# Autodesk Inventor assembly: SAR330  x 5 front + limit switches
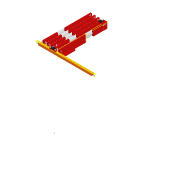
[picture p0: Inventor's stored thumbnail of the model, 180x180]
Saved by Autodesk Inventor 2020 (Build 240168000, 168)
## iProperties
Created: 2019-11-17
Part Number: SAR330  x 5 front + limit switches
Document SubType Name: Assembly
Designer: ball
Author: ball
## Documents named in this file (14)
- C:\FTC\FTC8863CAD\2019 Robot\Delivery\SAR330  x 5 front + limit switches.iam
- C:\FTC\FTC8863CAD\2019 Robot\Delivery\SAR330  x 5 + front couplers.iam
- C:\FTC\FTC8863CAD\Actobotics\605 parts\605630.ipt
- C:\FTC\FTC8863CAD\2019 Robot\Delivery\Coupler receiver.ipt
- C:\FTC\FTC8863CAD\RevRobotics\REV-41-1017_15mm_extrusion_17.875in.ipt
- C:\FTC\FTC8863CAD\StepLibraries\Screws\M3x6 SOCKET HEAD CAP SCREW.ipt
- C:\FTC\FTC8863CAD\2019 Robot\Delivery\Limit switch mount top.ipt
- C:\FTC\FTC8863CAD\2019 Robot\Delivery\Limit swtich mount bottom.ipt
- C:\FTC\FTC8863CAD\StepLibraries\Nuts\2-56 NYLON-INSERT LOCKNUT.ipt
- C:\FTC\FTC8863CAD\StepLibraries\Screws\2-56 x 0_5 SOCKET HEAD CAP SCREW.ipt
- C:\FTC\FTC8863CAD\StepLibraries\Nuts\m3 18-8 STAINLESS STL NYLON-INSERT LOCKNUT.ipt
- C:\FTC\FTC8863CAD\StepLibraries\Screws\M3 x 12 HEX HEAD CAP SCREW.ipt
- C:\FTC\FTC8863CAD\StepLibraries\Screws\M3 x 25 HEX HEAD CAP SCREW.ipt
- C:\FTC\FTC8863CAD\2019 Robot\Delivery\Limit switch mount top front.ipt
## Components (19 placed, 13 different names)
1. SAR330  x 5 + front couplers:1 [sub-assembly] — Flush:1, Flush:2, Mate:1, Mate:2, Flush:3, Flush:4, Mate:3, Flush:5, Flush:6, Mate:5, Flush:7, Mate:6, Flush:8, Flush:9, Mate:18, Mate:19, Flush:13, Mate:20, Flush:14, Flush:15
2. 605630:1 — Flush:1, Flush:2, Mate:1
3. Coupler receiver:1 — Mate:2, Flush:3, Flush:4
4. REV-41-1017_15mm_extrusion_17.875in:1 — Mate:3, Flush:5, Flush:6, Mate:4, Flush:10, Flush:11, Flush:12, Mate:16
5. 605630:2 — Mate:4, Mate:5, Flush:7, Mate:9, Mate:10, Mate:11
6. M3x6 SOCKET HEAD CAP SCREW:3 — Mate:6
7. Limit switch mount top:1 — Flush:8, Flush:9
8. Limit swtich mount bottom:1 — Flush:10, Flush:11, Flush:12, Mate:8, Mate:12, Mate:13, Mate:14, Mate:15
9. 2-56 NYLON-INSERT LOCKNUT:1
10. 2-56 NYLON-INSERT LOCKNUT:2 — Mate:8, Mate:9
11. 2-56 x 0_5 SOCKET HEAD CAP SCREW:1 — Mate:10, Mate:11
12. m3 18-8 STAINLESS STL NYLON-INSERT LOCKNUT:1 — Mate:12, Mate:13, Mate:17
13. m3 18-8 STAINLESS STL NYLON-INSERT LOCKNUT:2 — Mate:14, Mate:15
14. M3 x 12 HEX HEAD CAP SCREW:1 — Mate:16, Mate:17
15. 605630:3 — Flush:13, Mate:20, Flush:14, Mate:21, Mate:24
16. M3 x 25 HEX HEAD CAP SCREW:1 — Mate:18, Mate:19
17. Limit switch mount top front:1 — Flush:15, Mate:22
18. 2-56 x 0_5 SOCKET HEAD CAP SCREW:2 — Mate:21, Mate:22, Mate:23
19. 2-56 NYLON-INSERT LOCKNUT:3 — Mate:23, Mate:24
## Relationships (39: Mate 24, Flush 15)
- Flush:1 (14.605 mm): SAR330  x 5 + front couplers:1 ↔ 605630:1
- Flush:2 (10.16 mm): SAR330  x 5 + front couplers:1 ↔ 605630:1
- Mate:1 (2.8702 mm): SAR330  x 5 + front couplers:1 ↔ 605630:1
- Mate:2: SAR330  x 5 + front couplers:1 ↔ Coupler receiver:1
- Flush:3: SAR330  x 5 + front couplers:1 ↔ Coupler receiver:1
- Flush:4: SAR330  x 5 + front couplers:1 ↔ Coupler receiver:1
- Mate:3: SAR330  x 5 + front couplers:1 ↔ REV-41-1017_15mm_extrusion_17.875in:1
- Flush:5: SAR330  x 5 + front couplers:1 ↔ REV-41-1017_15mm_extrusion_17.875in:1
- Flush:6: SAR330  x 5 + front couplers:1 ↔ REV-41-1017_15mm_extrusion_17.875in:1
- Mate:4 (6.985 mm): REV-41-1017_15mm_extrusion_17.875in:1 ↔ 605630:2
- Mate:5 (1.27 mm): SAR330  x 5 + front couplers:1 ↔ 605630:2
- Flush:7: SAR330  x 5 + front couplers:1 ↔ 605630:2
- Mate:6 (2.286 mm): SAR330  x 5 + front couplers:1 ↔ M3x6 SOCKET HEAD CAP SCREW:3
- [Mate]: SAR330  x 5 + front couplers:1 ↔ M3x6 SOCKET HEAD CAP SCREW:3
- Flush:8: SAR330  x 5 + front couplers:1 ↔ Limit switch mount top:1
- Flush:9: SAR330  x 5 + front couplers:1 ↔ Limit switch mount top:1
- Flush:10: REV-41-1017_15mm_extrusion_17.875in:1 ↔ Limit swtich mount bottom:1
- Flush:11: REV-41-1017_15mm_extrusion_17.875in:1 ↔ Limit swtich mount bottom:1
- Flush:12: REV-41-1017_15mm_extrusion_17.875in:1 ↔ Limit swtich mount bottom:1
- Mate:8: Limit swtich mount bottom:1 ↔ 2-56 NYLON-INSERT LOCKNUT:2
- Mate:9: 605630:2 ↔ 2-56 NYLON-INSERT LOCKNUT:2
- Mate:10: 605630:2 ↔ 2-56 x 0_5 SOCKET HEAD CAP SCREW:1
- Mate:11: 605630:2 ↔ 2-56 x 0_5 SOCKET HEAD CAP SCREW:1
- Mate:12: Limit swtich mount bottom:1 ↔ m3 18-8 STAINLESS STL NYLON-INSERT LOCKNUT:1
- Mate:13: Limit swtich mount bottom:1 ↔ m3 18-8 STAINLESS STL NYLON-INSERT LOCKNUT:1
- Mate:14: Limit swtich mount bottom:1 ↔ m3 18-8 STAINLESS STL NYLON-INSERT LOCKNUT:2
- Mate:15: Limit swtich mount bottom:1 ↔ m3 18-8 STAINLESS STL NYLON-INSERT LOCKNUT:2
- Mate:16: REV-41-1017_15mm_extrusion_17.875in:1 ↔ M3 x 12 HEX HEAD CAP SCREW:1
- Mate:17: m3 18-8 STAINLESS STL NYLON-INSERT LOCKNUT:1 ↔ M3 x 12 HEX HEAD CAP SCREW:1
- Mate:18: SAR330  x 5 + front couplers:1 ↔ M3 x 25 HEX HEAD CAP SCREW:1
- Mate:19 (6 mm): SAR330  x 5 + front couplers:1 ↔ M3 x 25 HEX HEAD CAP SCREW:1
- Flush:13 (10.16 mm): SAR330  x 5 + front couplers:1 ↔ 605630:3
- Mate:20 (2.54 mm): SAR330  x 5 + front couplers:1 ↔ 605630:3
- Flush:14 (9 mm): SAR330  x 5 + front couplers:1 ↔ 605630:3
- Flush:15: SAR330  x 5 + front couplers:1 ↔ Limit switch mount top front:1
- Mate:21: 605630:3 ↔ 2-56 x 0_5 SOCKET HEAD CAP SCREW:2
- Mate:22: Limit switch mount top front:1 ↔ 2-56 x 0_5 SOCKET HEAD CAP SCREW:2
- Mate:23: 2-56 x 0_5 SOCKET HEAD CAP SCREW:2 ↔ 2-56 NYLON-INSERT LOCKNUT:3
- Mate:24: 605630:3 ↔ 2-56 NYLON-INSERT LOCKNUT:3
